# Autodesk Inventor assembly: Assembly 1
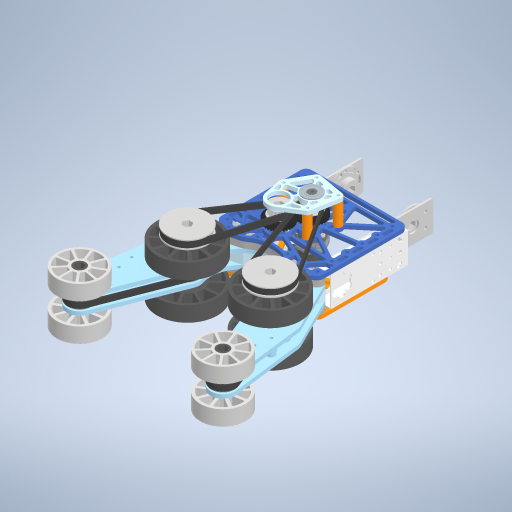
[picture p0: Inventor's stored thumbnail of the model, 512x512]
Saved by Autodesk Inventor 2023 (Build 270158000, 158)
## iProperties
Created: 2023-03-20
Part Number: Assembly 1
Description: STEP AP242
Document SubType Name: Assembly
Designer: Gabriel - T3 CAD
Preprocessor: ST-DEVELOPER v18.102
Title: 6417ddd0688ff71abd295de7
## Documents named in this file (27)
- C:\Users\Gabriel - T3 CAD\Documents\GitHub\T3-CAD\Stock\STOLEN GRIPPER-INTAKE MIX\Assembly 1 (1).iam
- C:\Users\Gabriel - T3 CAD\Downloads\Part 15.ipt
- C:\Users\Gabriel - T3 CAD\Downloads\4_ OD 1_2_ Hex Bore Compliant Wheel 35A (am-3480).ipt
- C:\Users\Gabriel - T3 CAD\Downloads\.5_ Hex ID 1.125_ OD Flanged Bearing (217-2734).ipt
- C:\Users\Gabriel - T3 CAD\Downloads\am-3946 3IN 500Hex Molded Compliant Wheel VER 2.ipt
- C:\Users\Gabriel - T3 CAD\Downloads\am-3946 3IN 500Hex Molded Compliant Wheel VER 2_1.ipt
- C:\Users\Gabriel - T3 CAD\Downloads\1_4_ 1_2_ Hex Acetal Spacer (217-3259).ipt
- C:\Users\Gabriel - T3 CAD\Downloads\18t 9mm Wide 1_2_ Hex Bore Double Flange 5mm HTD Aluminum Pulley (217-3225).ipt
- C:\Users\Gabriel - T3 CAD\Downloads\1_16_ 1_2_ Hex Acetal Spacer (217-3257).ipt
- C:\Users\Gabriel - T3 CAD\Downloads\24T HTD Pulley 10mm Wide.ipt
- C:\Users\Gabriel - T3 CAD\Downloads\76t 5mm Belt.ipt
- C:\Users\Gabriel - T3 CAD\Downloads\Part 7.ipt
- C:\Users\Gabriel - T3 CAD\Downloads\6328-23-P-0307.ipt
- C:\Users\Gabriel - T3 CAD\Downloads\Part 6.ipt
- C:\Users\Gabriel - T3 CAD\Downloads\THE TUBE YEAH.ipt
- C:\Users\Gabriel - T3 CAD\Downloads\Part 10.ipt
- C:\Users\Gabriel - T3 CAD\Downloads\32T 20DP Steel - 1_2_ Hex Bore Gear (REV-21-1927).ipt
- C:\Users\Gabriel - T3 CAD\Downloads\80t 5mm Belt.ipt
- C:\Users\Gabriel - T3 CAD\Downloads\Part 3.ipt
- C:\Users\Gabriel - T3 CAD\Downloads\Part 1.ipt
- C:\Users\Gabriel - T3 CAD\Downloads\Part 2.ipt
- C:\Users\Gabriel - T3 CAD\Downloads\Tube 2_x1_x5.116_.ipt
- C:\Users\Gabriel - T3 CAD\Downloads\92t 5mm Belt.ipt
- C:\Users\Gabriel - T3 CAD\Downloads\Part 14.ipt
- C:\Users\Gabriel - T3 CAD\Downloads\REV Ultraplanetary (Configurable) _1_.iam
- C:\Users\Gabriel - T3 CAD\Documents\GitHub\T3-CAD\Stock\Versa System\1_2” Hex Bore Aluminum VersaHub (217-2592).ipt
- C:\Users\Gabriel - T3 CAD\Downloads\Part3.ipt
## Components (76 placed, 74 different names)
1. NAUO1
2. NAUO2
3. NAUO3
4. NAUO4
5. NAUO5
6. NAUO6
7. NAUO7
8. NAUO8
9. NAUO9
10. NAUO10
11. NAUO11
12. NAUO12
13. NAUO13
14. NAUO14
15. NAUO15
16. NAUO16
17. NAUO17
18. NAUO18
19. NAUO19
20. NAUO20
21. NAUO21
22. NAUO22
23. NAUO23
24. NAUO24
25. NAUO25 — Rotational:7, Rotational:8
26. NAUO26
27. NAUO27
28. NAUO28
29. NAUO29
30. NAUO30
31. NAUO31
32. NAUO32
33. NAUO33
34. NAUO34
35. NAUO35
36. NAUO36
37. NAUO37
38. NAUO38
39. NAUO39
40. NAUO40
41. NAUO41
42. NAUO42
43. NAUO43
44. NAUO44
45. NAUO45
46. NAUO46
47. NAUO47
48. NAUO48
49. NAUO49 — Rotational:5, Rotational:6
50. NAUO50
51. NAUO51
52. NAUO52
53. NAUO53
54. NAUO54
55. NAUO55
56. NAUO56
57. NAUO57
58. NAUO58
59. NAUO59
60. NAUO60
61. NAUO61
62. NAUO62
63. NAUO63
64. NAUO64
65. NAUO65
66. NAUO66
67. NAUO67
68. NAUO68
69. NAUO69
70. NAUO70
71. NAUO118 [sub-assembly]
72. NAUO119
73. Part3:1 — Rotational:1, Rotational:2, Rotational:7, Rotational:8
74. Part3:2 — Rotational:3, Rotational:4, Rotational:5, Rotational:6
75. 1_2” Hex Bore Aluminum VersaHub (217-2592):3 — Rotational:1, Rotational:2
76. 1_2” Hex Bore Aluminum VersaHub (217-2592):4 — Rotational:3, Rotational:4
## Relationships (8: RevoluteJoint 8)
- Rotational:1 [RevoluteJoint]: Part3:1 ↔ 1_2” Hex Bore Aluminum VersaHub (217-2592):3
- Rotational:2 [RevoluteJoint]: Part3:1 ↔ 1_2” Hex Bore Aluminum VersaHub (217-2592):3
- Rotational:3 [RevoluteJoint]: Part3:2 ↔ 1_2” Hex Bore Aluminum VersaHub (217-2592):4
- Rotational:4 [RevoluteJoint]: Part3:2 ↔ 1_2” Hex Bore Aluminum VersaHub (217-2592):4
- Rotational:5 [RevoluteJoint]: NAUO49 ↔ Part3:2
- Rotational:6 [RevoluteJoint]: NAUO49 ↔ Part3:2
- Rotational:7 [RevoluteJoint]: NAUO25 ↔ Part3:1
- Rotational:8 [RevoluteJoint]: NAUO25 ↔ Part3:1
